# Autodesk Inventor assembly: Electronics Endcap Port Assembly
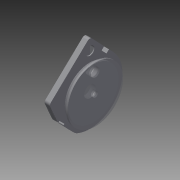
[picture p0: Inventor's stored thumbnail of the model, 180x180]
Saved by Autodesk Inventor 2015 (Build 190159000, 159)
## iProperties
Created: 2015-01-14
Part Number: Electronics Endcap Port Assembly
Document SubType Name: Assembly
Designer: Stackpole
Author: Stackpole
## Documents named in this file (6)
- C:\Users\Stackpole\Desktop\Brian G\V2.7\Electronics Tube\Electronics Endcaps\Electronics Endcap Port Assembly.iam
- C:\Users\Stackpole\Desktop\Brian G\V2.7\Electronics Tube\Electronics Endcaps\Electronics Endcaps Outer Gland Wall.ipt
- C:\Users\Stackpole\Desktop\Brian G\V2.7\Electronics Tube\Electronics Endcaps\Electronics Endcaps Inner Gland.ipt
- C:\Users\Stackpole\Desktop\Brian G\V2.7\Electronics Tube\Electronics Endcaps\Electronics Endcaps Inner Flange.ipt
- C:\Users\Stackpole\Desktop\Brian G\V2.7\Electronics Tube\Electronics Endcaps\Electronics Endcaps Middle Flange.ipt
- C:\Users\Stackpole\Desktop\Brian G\V2.7\Electronics Tube\Electronics Endcaps\Electronics Endcaps Outer Flange.ipt
## Components (5 placed, 5 different names)
1. Electronics Endcaps Outer Gland Wall:1 — Mate:1, Mate:2, Mate:3, Mate:5, Mate:6
2. Electronics Endcaps Inner Gland:1 — Mate:1, Mate:2, Mate:3, Mate:4
3. Electronics Endcaps Inner Flange:1 — Mate:4, Mate:5, Mate:6, Mate:7, Flush:1, Flush:2
4. Electronics Endcaps Middle Flange:1 — Mate:7, Flush:1, Flush:2, Mate:8, Flush:3, Flush:4
5. Electronics Endcaps Outer Flange:1 — Mate:8, Flush:3, Flush:4
## Relationships (12: Mate 8, Flush 4)
- Mate:1: Electronics Endcaps Outer Gland Wall:1 ↔ Electronics Endcaps Inner Gland:1
- Mate:2: Electronics Endcaps Outer Gland Wall:1 ↔ Electronics Endcaps Inner Gland:1
- Mate:3: Electronics Endcaps Outer Gland Wall:1 ↔ Electronics Endcaps Inner Gland:1
- Mate:4: Electronics Endcaps Inner Gland:1 ↔ Electronics Endcaps Inner Flange:1
- Mate:5: Electronics Endcaps Outer Gland Wall:1 ↔ Electronics Endcaps Inner Flange:1
- Mate:6: Electronics Endcaps Outer Gland Wall:1 ↔ Electronics Endcaps Inner Flange:1
- Mate:7: Electronics Endcaps Inner Flange:1 ↔ Electronics Endcaps Middle Flange:1
- Flush:1: Electronics Endcaps Inner Flange:1 ↔ Electronics Endcaps Middle Flange:1
- Flush:2: Electronics Endcaps Inner Flange:1 ↔ Electronics Endcaps Middle Flange:1
- Mate:8: Electronics Endcaps Middle Flange:1 ↔ Electronics Endcaps Outer Flange:1
- Flush:3: Electronics Endcaps Middle Flange:1 ↔ Electronics Endcaps Outer Flange:1
- Flush:4: Electronics Endcaps Middle Flange:1 ↔ Electronics Endcaps Outer Flange:1
